# Autodesk Inventor assembly: Ensamble - Jorge Paz - 1129421
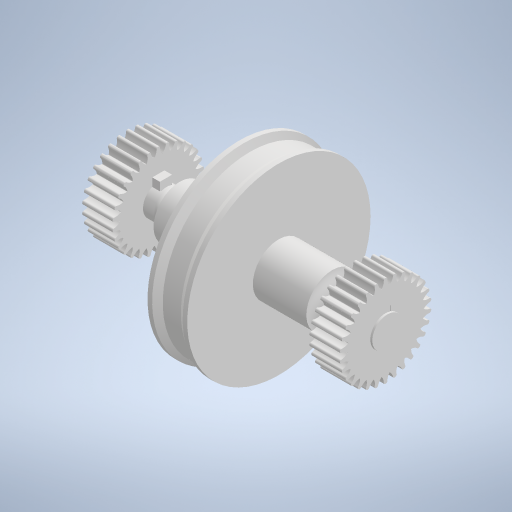
[picture p0: Inventor's stored thumbnail of the model, 512x512]
Saved by Autodesk Inventor 2024 (Build 280153000, 153)
## iProperties
Created: 2024-03-30
Part Number: Ensamble - Jorge Paz - 1129421
Document SubType Name: Assembly
Designer: pazjo
Author: pazjo
## Documents named in this file (5)
- C:\Users\pazjo\OneDrive\Escritorio\Ensamble - Jorge Paz - 1129421.iam
- C:\Users\pazjo\OneDrive\Escritorio\POLEA.ipt
- C:\Users\pazjo\OneDrive\Escritorio\CUÑA.ipt
- C:\Users\pazjo\OneDrive\Escritorio\EJE_CUÑEROS.ipt
- C:\Users\pazjo\OneDrive\Escritorio\ENGRANE.ipt
## Components (6 placed, 4 different names)
1. POLEA:1 — Insertar:1
2. EJE_CUÑEROS:1 — Insertar:1, Rígido:1, Insertar:2, Coincidencia:1
3. CUÑA:5 — Rígido:1
4. ENGRANE:2 — Insertar:2
5. ENGRANE:3 — Coincidencia:1, Rígido:2
6. CUÑA:6 — Rígido:2
## Relationships (5: Insert 2, WeldJoint 2, Mate 1)
- Insertar:1 (-35 mm): POLEA:1 ↔ EJE_CUÑEROS:1
- Rígido:1 [WeldJoint]: EJE_CUÑEROS:1 ↔ CUÑA:5
- Insertar:2 (0.5 mm): EJE_CUÑEROS:1 ↔ ENGRANE:2
- Coincidencia:1 [Mate]: EJE_CUÑEROS:1 ↔ ENGRANE:3
- Rígido:2 [WeldJoint]: ENGRANE:3 ↔ CUÑA:6
